# Autodesk Inventor assembly: full
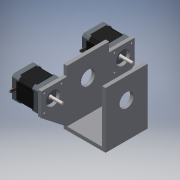
[picture p0: Inventor's stored thumbnail of the model, 180x180]
Saved by Autodesk Inventor 2019 (Build 230136000, 136)
## iProperties
Created: 2019-02-20
Part Number: full
Document SubType Name: Assembly
Designer: s-2508366
Author: s-2508366
## Documents named in this file (3)
- C:\Users\s-2508366\workspace\fbd-brachium\cad\full.iam
- C:\Users\s-2508366\workspace\fbd-brachium\cad\shoulder.ipt
- C:\Users\s-2508366\workspace\fbd-brachium\cad\Nema17.ipt
## Components (3 placed, 2 different names)
1. shoulder:1 — Insert:1, Insert:2, Insert:3, Insert:4
2. Nema17:2 — Insert:1, Insert:2
3. Nema17:3 — Insert:3, Insert:4
## Relationships (4: Insert 4)
- Insert:1: shoulder:1 ↔ Nema17:2
- Insert:2: shoulder:1 ↔ Nema17:2
- Insert:3: shoulder:1 ↔ Nema17:3
- Insert:4: shoulder:1 ↔ Nema17:3
